# Autodesk Inventor assembly: Propeller_complete
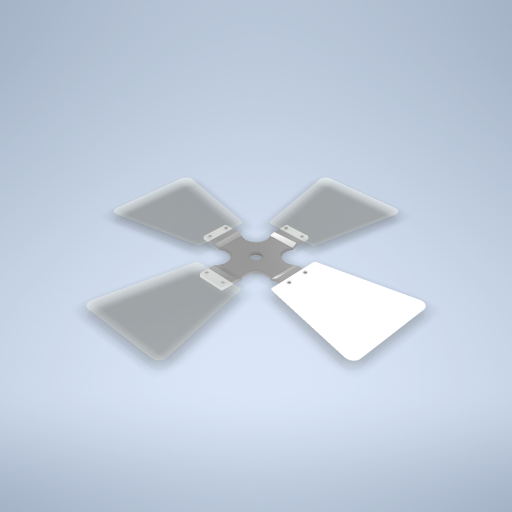
[picture p0: Inventor's stored thumbnail of the model, 512x512]
Saved by Autodesk Inventor 2024.2 (Build 282272000, 272)
## iProperties
Created: 2024-05-14
Part Number: Propeller_complete
Document SubType Name: Assembly
Designer: Fabri
Author: Fabri
## Documents named in this file (3)
- C:\Users\Fabri\Documents\Inventor\Stirlingfan\Propeller_complete.iam
- C:\Users\Fabri\Documents\Inventor\Stirlingfan\propeller.ipt
- C:\Users\Fabri\Documents\Inventor\Stirlingfan\propeller_extensions.ipt
## Components (5 placed, 2 different names)
1. propeller:1 — Passend:1, Drehbar:1, Passend:2, Passend:3, Passend:4, Drehbar:2, Drehbar:3, Drehbar:4
2. propeller_extensions:1 — Passend:1, Drehbar:1
3. propeller_extensions:2 — Passend:2, Drehbar:2
4. propeller_extensions:3 — Passend:3, Drehbar:3
5. propeller_extensions:4 — Passend:4, Drehbar:4
## Relationships (8: Mate 4, RevoluteJoint 4)
- Passend:1 [Mate]: propeller:1 ↔ propeller_extensions:1
- Drehbar:1 [RevoluteJoint]: propeller:1 ↔ propeller_extensions:1
- Passend:2 [Mate]: propeller:1 ↔ propeller_extensions:2
- Passend:3 [Mate]: propeller:1 ↔ propeller_extensions:3
- Passend:4 [Mate]: propeller:1 ↔ propeller_extensions:4
- Drehbar:2 [RevoluteJoint]: propeller:1 ↔ propeller_extensions:2
- Drehbar:3 [RevoluteJoint]: propeller:1 ↔ propeller_extensions:3
- Drehbar:4 [RevoluteJoint]: propeller:1 ↔ propeller_extensions:4
